# Autodesk Inventor assembly: LiftMechanism
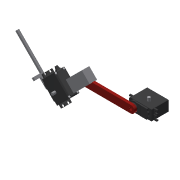
[picture p0: Inventor's stored thumbnail of the model, 180x180]
Saved by Autodesk Inventor 2018 (Build 220112000, 112)
## iProperties
Created: 2018-09-24
Part Number: LiftMechanism
Document SubType Name: Assembly
Designer: DCCUMD
Author: DCCUMD
## Documents named in this file (5)
- C:\Users\Vulnic\Desktop\School - Desktop\Fall 2018 Semester #1\ENES100\MS2 stuff\CAD FILES\LiftMechanism.iam
- C:\Users\Vulnic\Desktop\School - Desktop\Fall 2018 Semester #1\ENES100\MS2 stuff\CAD FILES\servo body.ipt
- C:\Users\Vulnic\Desktop\School - Desktop\Fall 2018 Semester #1\ENES100\MS2 stuff\CAD FILES\ServoConnector.ipt
- C:\Users\Vulnic\Desktop\School - Desktop\Fall 2018 Semester #1\ENES100\MS2 stuff\CAD FILES\Arms.ipt
- C:\Users\Vulnic\Desktop\School - Desktop\Fall 2018 Semester #1\ENES100\MS2 stuff\CAD FILES\ServoHolder.ipt
## Components (5 placed, 4 different names)
1. servo body:1 — Tangent:2, Mate:4
2. servo body:2 — Mate:3, Flush:5, Flush:6, Angle:1
3. ServoConnector:1 — Tangent:2, Mate:4, Angle:1, Flush:8, Angle:2
4. Arms:1 — Mate:3, Flush:5, Flush:6
5. ServoHolder:1 — Flush:8, Angle:2
## Relationships (8: Flush 3, Mate 2, Angle 2, Tangent 1)
- Mate:3: servo body:2 ↔ Arms:1
- Flush:5 (3 mm): servo body:2 ↔ Arms:1
- Flush:6 (-3 mm): servo body:2 ↔ Arms:1
- Tangent:2: servo body:1 ↔ ServoConnector:1
- Mate:4: servo body:1 ↔ ServoConnector:1
- Angle:1 (-45 deg): servo body:2 ↔ ServoConnector:1
- Flush:8 (-4.5 mm): ServoConnector:1 ↔ ServoHolder:1
- Angle:2 (-45 deg): ServoConnector:1 ↔ ServoHolder:1
